# Autodesk Inventor assembly: case
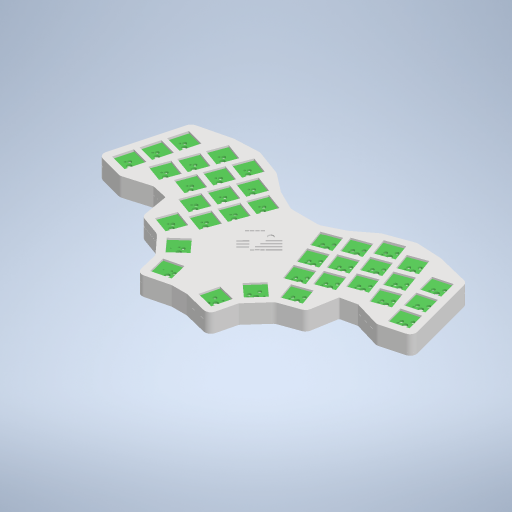
[picture p0: Inventor's stored thumbnail of the model, 512x512]
Saved by Autodesk Inventor 2024 (Build 280153000, 153)
## iProperties
Created: 2024-09-29
Part Number: case
Document SubType Name: Assembly
Designer: nikla
Author: nikla
## Documents named in this file (4)
- C:\Users\nikla\OneDrive\Keyboards\Blavinge\case\1-part\case.iam
- C:\Users\nikla\OneDrive\Keyboards\Blavinge\kicad\blavinge\blavinge.iam
- C:\Users\nikla\OneDrive\Keyboards\Blavinge\case\1-part\bottom.ipt
- C:\Users\nikla\OneDrive\Keyboards\Blavinge\case\1-part\top.ipt
## Components (3 placed, 3 different names)
1. blavinge:1 [sub-assembly] — Passend:1, Passend:2, Passend:3, Passend:4
2. bottom:1 — Fluchtend:1, Fluchtend:2, Passend:4
3. top:1 — Passend:1, Passend:2, Passend:3, Fluchtend:1, Fluchtend:2
## Relationships (6: Mate 4, Flush 2)
- Passend:1 [Mate]: blavinge:1 ↔ top:1
- Passend:2 [Mate]: blavinge:1 ↔ top:1
- Passend:3 [Mate]: blavinge:1 ↔ top:1
- Fluchtend:1 [Flush]: bottom:1 ↔ top:1
- Fluchtend:2 [Flush]: bottom:1 ↔ top:1
- Passend:4 [Mate]: blavinge:1 ↔ bottom:1
